# Autodesk Inventor assembly: case
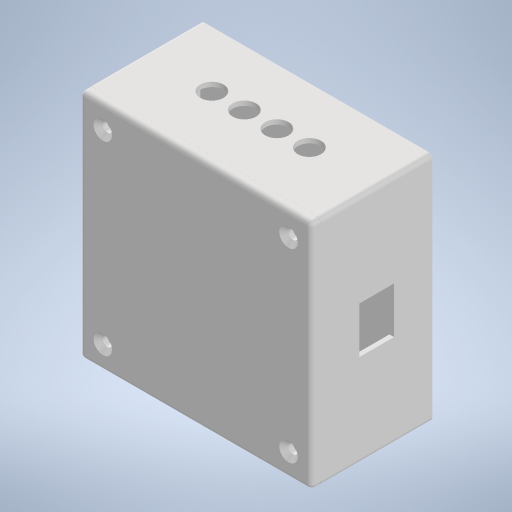
[picture p0: Inventor's stored thumbnail of the model, 512x512]
Saved by Autodesk Inventor 2023 (Build 270158000, 158)
## iProperties
Created: 2023-05-04
Part Number: case
Document SubType Name: Assembly
Designer: cocqu
Author: cocqu
## Documents named in this file (3)
- C:\Projects\sem2\projectwerk\low-voltage-UPS\case\inventor\case.iam
- C:\Projects\sem2\projectwerk\low-voltage-UPS\case\inventor\Base.ipt
- C:\Projects\sem2\projectwerk\low-voltage-UPS\case\inventor\Lid.ipt
## Components (2 placed, 2 different names)
1. Base:1 — Mate:1, Flush:1, Flush:2
2. Lid:1 — Mate:1, Flush:1, Flush:2
## Relationships (3: Flush 2, Mate 1)
- Mate:1: Base:1 ↔ Lid:1
- Flush:1: Base:1 ↔ Lid:1
- Flush:2: Base:1 ↔ Lid:1
